# Autodesk Inventor assembly: Assembly15
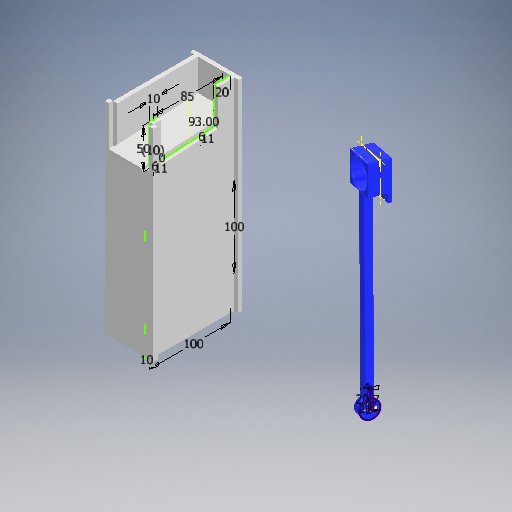
[picture p0: Inventor's stored thumbnail of the model, 512x512]
Saved by Autodesk Inventor 2025.3 (Build 293356000, 356)
## iProperties
Created: 2026-04-09
Part Number: Assembly15
Document SubType Name: Assembly
Designer: user
Author: user
## Documents named in this file (4)
- C:\Ayman\Inventor Projects\Lifting Mechanism\Assembly15.iam
- C:\Ayman\Inventor Projects\Lifting Mechanism\arm.ipt
- C:\Ayman\Inventor Projects\Lifting Mechanism\Assembly2 22.iam
- C:\Ayman\Inventor Projects\Lifting Mechanism\Lifting Sections floor.ipt
## Components (3 placed, 3 different names)
1. arm:1
2. Assembly2 22:1 [sub-assembly] — Mate:1, Mate:2
3. Lifting Sections floor:1 — Mate:1, Mate:2
## Relationships (2: Mate 2)
- Mate:1: Assembly2 22:1 ↔ Lifting Sections floor:1
- Mate:2: Assembly2 22:1 ↔ Lifting Sections floor:1
